# Autodesk Inventor assembly: HexAxelWithCamTilt
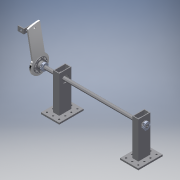
[picture p0: Inventor's stored thumbnail of the model, 180x180]
Saved by Autodesk Inventor 2017 (Build 210142000, 142)
## iProperties
Created: 2016-05-18
Part Number: HexAxelWithCamTilt
Document SubType Name: Assembly
Designer: steele
Author: steele
## Documents named in this file (8)
- C:\snobotics\CAD-Development\robSteele\SnoBotics2016\2016-05-05-ShooterPrototype\HexAxelWithCamTilt.iam
- C:\snobotics\CAD-Development\robSteele\SnoBotics2016\2016-05-05-ShooterPrototype\PostForHexAxel.ipt
- C:\snobotics\CAD-MfgResources\VexRobotics\ThunderHex\217-4396FlangedBearing.ipt
- C:\snobotics\CAD-MfgResources\VexRobotics\ThunderHex\217-4002-Hex_1_2x18inch.ipt
- C:\snobotics\CAD-MfgResources\VexRobotics\ThunderHex\217-4106-HiStrengthClampingCollar.iam
- C:\snobotics\CAD-MfgResources\VexRobotics\ThunderHex\217-2592-VersaHub_1_2_inch.ipt
- C:\snobotics\CAD-Development\robSteele\SnoBotics2016\2016-05-05-ShooterPrototype\camPlateCircular.ipt
- C:\snobotics\CAD-Development\robSteele\SnoBotics2016\2016-05-05-ShooterPrototype\simpleBracketForTopOfDart.ipt
## Components (12 placed, 7 different names)
1. PostForHexAxel:1 — Flush:1, Flush:2, Mate:1, Insert:1
2. PostForHexAxel:2 — Flush:1, Flush:2, Mate:1, Insert:2
3. 217-4396FlangedBearing:1 — Insert:1, Insert:3, Insert:10
4. 217-4396FlangedBearing:2 — Insert:2, Insert:4
5. 217-4002-Hex_1_2x18inch:1 — Insert:3, Insert:5
6. 217-4106-HiStrengthClampingCollar:1 [sub-assembly] — Insert:4
7. 217-2592-VersaHub_1_2_inch:1 — Insert:5, Insert:6, Insert:7, Insert:8, Insert:9
8. camPlateCircular:1 — Insert:6, Insert:7, Insert:11
9. 217-4106-HiStrengthClampingCollar:2 [sub-assembly] — Insert:8
10. 217-4106-HiStrengthClampingCollar:3 [sub-assembly] — Insert:9
11. 217-4106-HiStrengthClampingCollar:4 [sub-assembly] — Insert:10
12. simpleBracketForTopOfDart:1 — Insert:11
## Relationships (14: Insert 11, Flush 2, Mate 1)
- Flush:1: PostForHexAxel:1 ↔ PostForHexAxel:2
- Flush:2: PostForHexAxel:1 ↔ PostForHexAxel:2
- Mate:1 (304.8 mm): PostForHexAxel:1 ↔ PostForHexAxel:2
- Insert:1: PostForHexAxel:1 ↔ 217-4396FlangedBearing:1
- Insert:2: PostForHexAxel:2 ↔ 217-4396FlangedBearing:2
- Insert:3 (87.63 mm): 217-4396FlangedBearing:1 ↔ 217-4002-Hex_1_2x18inch:1
- Insert:4: 217-4396FlangedBearing:2 ↔ 217-4106-HiStrengthClampingCollar:1
- Insert:5 (-9.525 mm): 217-4002-Hex_1_2x18inch:1 ↔ 217-2592-VersaHub_1_2_inch:1
- Insert:6: 217-2592-VersaHub_1_2_inch:1 ↔ camPlateCircular:1
- Insert:7: 217-2592-VersaHub_1_2_inch:1 ↔ camPlateCircular:1
- Insert:8: 217-2592-VersaHub_1_2_inch:1 ↔ 217-4106-HiStrengthClampingCollar:2
- Insert:9: 217-2592-VersaHub_1_2_inch:1 ↔ 217-4106-HiStrengthClampingCollar:3
- Insert:10: 217-4396FlangedBearing:1 ↔ 217-4106-HiStrengthClampingCollar:4
- Insert:11: camPlateCircular:1 ↔ simpleBracketForTopOfDart:1
